# Autodesk Inventor assembly: S13360-13xxPE
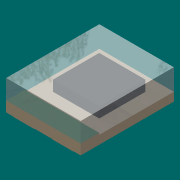
[picture p0: Inventor's stored thumbnail of the model, 180x180]
Saved by Autodesk Inventor 2016 (Build 200138000, 138)
## iProperties
Created: 2016-03-28
Part Number: S13360-13xxPE
Document SubType Name: Assembly
Designer: sawai
Author: sawai
## Documents named in this file (3)
- C:\Users\Jonathan\Documents\Projects\loop\scintillatorPanel\dependency\mppcSensorInterface\cad\electronics\S13360-13xxPE\S13360-13xxPE.iam
- C:\Users\Jonathan\Documents\Projects\loop\scintillatorPanel\dependency\mppcSensorInterface\cad\electronics\S13360-13xxPE\mppc.ipt
- C:\Users\Jonathan\Documents\Projects\loop\scintillatorPanel\dependency\mppcSensorInterface\cad\electronics\S13360-13xxPE\epoxy.ipt
## Components (2 placed, 2 different names)
1. mppc:1 — Flush:1
2. epoxy:1 — Flush:1
## Relationships (1: Flush 1)
- Flush:1: mppc:1 ↔ epoxy:1
